# Autodesk Inventor assembly: robotassembly1
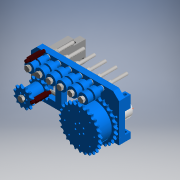
[picture p0: Inventor's stored thumbnail of the model, 180x180]
Saved by Autodesk Inventor 2016 (Build 200138000, 138)
## iProperties
Created: 2016-05-14
Part Number: robotassembly1
Document SubType Name: Assembly
Designer: hesaon
Author: hesaon
## Documents named in this file (21)
- C:\Users\hesaon\Documents\Killer-Bot-2016\AutodeskWorkspace\robotassembly1.iam
- C:\Users\hesaon\Documents\Killer-Bot-2016\AutodeskWorkspace\motorHolder57mmVer2.ipt
- C:\Users\hesaon\Documents\Killer-Bot-2016\AutodeskWorkspace\37D mm metal gearmotor.ipt
- C:\Users\hesaon\Documents\Killer-Bot-2016\AutodeskWorkspace\mountingHub6mm.ipt
- C:\Users\hesaon\Documents\Killer-Bot-2016\AutodeskWorkspace\sprocketsHolder.ipt
- C:\Users\hesaon\Documents\Killer-Bot-2016\AutodeskWorkspace\BigSprocket2.ipt
- C:\Users\hesaon\Documents\Killer-Bot-2016\AutodeskWorkspace\tracks_center.ipt
- C:\Users\hesaon\Documents\Killer-Bot-2016\AutodeskWorkspace\outerBigSprocket2.ipt
- C:\Users\hesaon\Documents\Killer-Bot-2016\AutodeskWorkspace\framesideRight.ipt
- C:\Users\hesaon\Documents\Killer-Bot-2016\AutodeskWorkspace\smallSprocketHolder.ipt
- C:\Users\hesaon\Documents\Killer-Bot-2016\AutodeskWorkspace\smallSprocket2.ipt
- C:\Users\hesaon\Documents\Killer-Bot-2016\AutodeskWorkspace\frameBack.ipt
- C:\Users\hesaon\Documents\Killer-Bot-2016\AutodeskWorkspace\pin5x60.ipt
- C:\Users\hesaon\Documents\Killer-Bot-2016\AutodeskWorkspace\smallSprocketFixture.ipt
- C:\Users\hesaon\Documents\Killer-Bot-2016\AutodeskWorkspace\roller.ipt
- C:\Users\hesaon\Documents\Killer-Bot-2016\AutodeskWorkspace\frameBottomRight.ipt
- C:\Users\hesaon\Documents\Killer-Bot-2016\AutodeskWorkspace\washer6mm.ipt
- C:\Users\hesaon\Documents\Killer-Bot-2016\AutodeskWorkspace\rollerdistance.ipt
- C:\Users\hesaon\Documents\Killer-Bot-2016\AutodeskWorkspace\nut6mm.ipt
- C:\Users\hesaon\Documents\Killer-Bot-2016\AutodeskWorkspace\bolt.ipt
- C:\Users\hesaon\Documents\Killer-Bot-2016\AutodeskWorkspace\battery.ipt
## Components (72 placed, 19 different names)
1. motorHolder57mmVer2:1 — Insert:1, Insert:2, Flush:2, Mate:5, Mate:6
2. 37D mm metal gearmotor:1 — Insert:1, Insert:2, Insert:3
3. mountingHub6mm:1 — Insert:3, Insert:9, Insert:10
4. sprocketsHolder:2 — Insert:7, Insert:8, Mate:1, Mate:2, Mate:3, Mate:4
5. Roller Chain Sprocket1:2 — Insert:7, Insert:8
6. Outer big sprocket:1 — Mate:1, Mate:2, Mate:3, Mate:4, Insert:9, Insert:10
7. framesideRight:1 — Flush:1, Insert:27, Insert:28, Flush:2, Mate:5, Mate:6, Insert:37, Flush:5, Flush:6, Flush:7, Mate:9
8. smallSprocketHolder:1 — Insert:13, Insert:14, Insert:15, Insert:16
9. Roller Chain Sprocket1:3 — Insert:13, Insert:14, Insert:93
10. Roller Chain Sprocket1:4 — Insert:15, Insert:16, Insert:17, Insert:92, Insert:94
11. tracks_center:2 — Insert:17
12. frameBack:1 — Flush:1, Flush:7
13. pin5x60:1 — Insert:27, Cylindrical:2
14. pin5x60:2 — Insert:28, Cylindrical:1
15. smallSprocketFixture:1 — Cylindrical:1, Cylindrical:2, Insert:91, Insert:95
16. roller:2 — Tangent:1, Flush:3, Flush:4, Insert:38, Insert:55, Insert:69
17. roller:3 — Insert:39, Insert:54, Insert:68
18. roller:4 — Insert:40, Insert:53, Insert:67
19. roller:5 — Insert:41, Insert:52, Insert:66
20. roller:6 — Insert:42, Insert:51, Insert:65
21. frameBottomRight:1 — Insert:37, Insert:38, Insert:39, Insert:40, Insert:41, Insert:42, Insert:43, Flush:5, Flush:6, Insert:44, Insert:45, Insert:46, Insert:47, Insert:48, Insert:49, Insert:71, Insert:72, Insert:73, Insert:74, Insert:75, Insert:76, Flush:8
22. tracks_center:3 — Tangent:1, Flush:3, Flush:4
23. roller:7 — Insert:43, Insert:50, Insert:64
24. washer6mm:1 — Insert:53
25. washer6mm:2 — Insert:51
26. washer6mm:3 — Insert:48, Insert:60
27. washer6mm:4 — Insert:47, Insert:59
28. washer6mm:5 — Insert:46, Insert:58
29. washer6mm:6 — Insert:49, Insert:61
30. washer6mm:7 — Insert:52
31. washer6mm:8 — Insert:44, Insert:56
32. washer6mm:9 — Insert:45, Insert:57
33. washer6mm:10 — Insert:55
34. washer6mm:11 — Insert:54
35. washer6mm:12 — Insert:50
36. rollerdistance:1 — Insert:61
37. rollerdistance:2 — Insert:59
38. rollerdistance:3 — Insert:60
39. rollerdistance:4 — Insert:58
40. rollerdistance:5 — Insert:57
41. rollerdistance:6 — Insert:56
42. nut6mm:1 — Insert:91, Insert:92, Insert:96
43. nut6mm:2 — Insert:90
44. nut6mm:3 — Insert:89
45. nut6mm:4 — Insert:88
46. nut6mm:5 — Insert:87
47. nut6mm:6 — Insert:86
48. nut6mm:7 — Insert:85
49. bolt:1 — Insert:80
50. bolt:2 — Insert:81
51. bolt:3 — Insert:82
52. bolt:4 — Insert:83
53. bolt:5 — Insert:97
54. bolt:6 — Insert:79
55. bolt:7 — Insert:78
56. washer6mm:13 — Insert:64, Insert:83
57. washer6mm:14 — Insert:65, Insert:82
58. washer6mm:15 — Insert:66, Insert:81
59. washer6mm:16 — Insert:67, Insert:80
60. washer6mm:17 — Insert:68, Insert:79
61. washer6mm:18 — Insert:69, Insert:78
62. washer6mm:19 — Insert:96
63. washer6mm:20 — Insert:93, Insert:97
64. washer6mm:21 — Insert:95
65. washer6mm:22 — Insert:94
66. washer6mm:23 — Insert:76, Insert:90
67. washer6mm:24 — Insert:72, Insert:86
68. washer6mm:25 — Insert:71, Insert:85
69. washer6mm:26 — Insert:75, Insert:89
70. washer6mm:27 — Insert:74, Insert:88
71. washer6mm:28 — Insert:73, Insert:87
72. battery:1 — Mate:9, Flush:8
## Relationships (88: Insert 70, Flush 8, Mate 7, CylindricalJoint 2, Tangent 1)
- Insert:1: motorHolder57mmVer2:1 ↔ 37D mm metal gearmotor:1
- Insert:2: motorHolder57mmVer2:1 ↔ 37D mm metal gearmotor:1
- Insert:3: 37D mm metal gearmotor:1 ↔ mountingHub6mm:1
- Insert:7: sprocketsHolder:2 ↔ Roller Chain Sprocket1:2
- Insert:8: sprocketsHolder:2 ↔ Roller Chain Sprocket1:2
- Mate:1: sprocketsHolder:2 ↔ Outer big sprocket:1
- Mate:2: sprocketsHolder:2 ↔ Outer big sprocket:1
- Mate:3: sprocketsHolder:2 ↔ Outer big sprocket:1
- Mate:4: sprocketsHolder:2 ↔ Outer big sprocket:1
- Insert:9: mountingHub6mm:1 ↔ Outer big sprocket:1
- Insert:10: mountingHub6mm:1 ↔ Outer big sprocket:1
- Insert:13: smallSprocketHolder:1 ↔ Roller Chain Sprocket1:3
- Insert:14: smallSprocketHolder:1 ↔ Roller Chain Sprocket1:3
- Insert:15: smallSprocketHolder:1 ↔ Roller Chain Sprocket1:4
- Insert:16: smallSprocketHolder:1 ↔ Roller Chain Sprocket1:4
- Insert:17: Roller Chain Sprocket1:4 ↔ tracks_center:2
- Flush:1: framesideRight:1 ↔ frameBack:1
- Insert:27: framesideRight:1 ↔ pin5x60:1
- Insert:28: framesideRight:1 ↔ pin5x60:2
- Flush:2: motorHolder57mmVer2:1 ↔ framesideRight:1
- Mate:5: motorHolder57mmVer2:1 ↔ framesideRight:1
- Tangent:1: roller:2 ↔ tracks_center:3
- Flush:3: roller:2 ↔ tracks_center:3
- Flush:4: roller:2 ↔ tracks_center:3
- Mate:6: motorHolder57mmVer2:1 ↔ framesideRight:1
- Insert:37: framesideRight:1 ↔ frameBottomRight:1
- Insert:38 (12.16 mm): roller:2 ↔ frameBottomRight:1
- Insert:39 (12.16 mm): roller:3 ↔ frameBottomRight:1
- Insert:40 (12.16 mm): roller:4 ↔ frameBottomRight:1
- Insert:41 (12.16 mm): roller:5 ↔ frameBottomRight:1
- Insert:42 (12.16 mm): roller:6 ↔ frameBottomRight:1
- Insert:43 (12.16 mm): frameBottomRight:1 ↔ roller:7
- Flush:5: framesideRight:1 ↔ frameBottomRight:1
- Flush:6: framesideRight:1 ↔ frameBottomRight:1
- Insert:44: frameBottomRight:1 ↔ washer6mm:8
- Insert:45: frameBottomRight:1 ↔ washer6mm:9
- Insert:46: frameBottomRight:1 ↔ washer6mm:5
- Insert:47: frameBottomRight:1 ↔ washer6mm:4
- Insert:48: frameBottomRight:1 ↔ washer6mm:3
- Insert:49: frameBottomRight:1 ↔ washer6mm:6
- Insert:50: roller:7 ↔ washer6mm:12
- Insert:51: roller:6 ↔ washer6mm:2
- Insert:52: roller:5 ↔ washer6mm:7
- Insert:53: roller:4 ↔ washer6mm:1
- Insert:54: roller:3 ↔ washer6mm:11
- Insert:55: roller:2 ↔ washer6mm:10
- Insert:56: washer6mm:8 ↔ rollerdistance:6
- Insert:57: washer6mm:9 ↔ rollerdistance:5
- Insert:58: washer6mm:5 ↔ rollerdistance:4
- Insert:59: washer6mm:4 ↔ rollerdistance:2
- Insert:60: washer6mm:3 ↔ rollerdistance:3
- Insert:61: washer6mm:6 ↔ rollerdistance:1
- Flush:7: framesideRight:1 ↔ frameBack:1
- Insert:64: roller:7 ↔ washer6mm:13
- Insert:65: roller:6 ↔ washer6mm:14
- Insert:66: roller:5 ↔ washer6mm:15
- Insert:67: roller:4 ↔ washer6mm:16
- Insert:68: roller:3 ↔ washer6mm:17
- Insert:69: roller:2 ↔ washer6mm:18
- Insert:71: frameBottomRight:1 ↔ washer6mm:25
- Insert:72: frameBottomRight:1 ↔ washer6mm:24
- Insert:73: frameBottomRight:1 ↔ washer6mm:28
- Insert:74: frameBottomRight:1 ↔ washer6mm:27
- Insert:75: frameBottomRight:1 ↔ washer6mm:26
- Insert:76: frameBottomRight:1 ↔ washer6mm:23
- Insert:78: bolt:7 ↔ washer6mm:18
- Insert:79: bolt:6 ↔ washer6mm:17
- Insert:80: bolt:1 ↔ washer6mm:16
- Insert:81: bolt:2 ↔ washer6mm:15
- Insert:82: bolt:3 ↔ washer6mm:14
- Insert:83: bolt:4 ↔ washer6mm:13
- Insert:85: nut6mm:7 ↔ washer6mm:25
- Insert:86: nut6mm:6 ↔ washer6mm:24
- Insert:87: nut6mm:5 ↔ washer6mm:28
- Insert:88: nut6mm:4 ↔ washer6mm:27
- Insert:89: nut6mm:3 ↔ washer6mm:26
- Insert:90: nut6mm:2 ↔ washer6mm:23
- Mate:9: framesideRight:1 ↔ battery:1
- Flush:8: frameBottomRight:1 ↔ battery:1
- Cylindrical:1: pin5x60:2 ↔ smallSprocketFixture:1
- Cylindrical:2: pin5x60:1 ↔ smallSprocketFixture:1
- Insert:91: smallSprocketFixture:1 ↔ nut6mm:1
- Insert:92 (11.5 mm): Roller Chain Sprocket1:4 ↔ nut6mm:1
- Insert:93: Roller Chain Sprocket1:3 ↔ washer6mm:20
- Insert:94: Roller Chain Sprocket1:4 ↔ washer6mm:22
- Insert:95: smallSprocketFixture:1 ↔ washer6mm:21
- Insert:96: nut6mm:1 ↔ washer6mm:19
- Insert:97: bolt:5 ↔ washer6mm:20
